# Autodesk Inventor assembly: CARRO
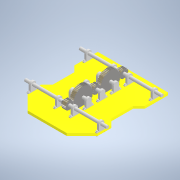
[picture p0: Inventor's stored thumbnail of the model, 180x180]
Saved by Autodesk Inventor 2021 (Build 250183000, 183)
## iProperties
Created: 2021-02-07
Part Number: CARRO
Document SubType Name: Assembly
Designer: rotje
Author: rotje
## Documents named in this file (5)
- C:\Users\rotje\Documents\Inventor\MSF\CARRO.iam
- C:\Users\rotje\Documents\Inventor\MSF\Base-soporte.iam
- C:\Users\rotje\Documents\Inventor\MSF\Eje-engrane.iam
- C:\Users\rotje\Documents\Inventor\MSF\Eje-engrane_chico.iam
- C:\Users\rotje\Documents\Inventor\MSF\Eje_Engrane-llanta.iam
## Components (6 placed, 4 different names)
1. Base-soporte:1 [sub-assembly] — Insertar:1, Insertar:2, Insertar:3, Coincidencia:1, Coincidencia:2, Coincidencia:3, Coincidencia:4
2. Eje-engrane:1 [sub-assembly] — Insertar:3, Nivelación:1, Tangente:3, Tangente:4, Rotación:3, Rotación:4
3. Eje-engrane:2 [sub-assembly] — Insertar:1, Nivelación:2, Tangente:1, Tangente:2, Rotación:1, Rotación:2
4. Eje-engrane_chico:1 [sub-assembly] — Insertar:2, Tangente:2, Tangente:3, Rotación:2, Rotación:3
5. Eje_Engrane-llanta:1 [sub-assembly] — Nivelación:1, Coincidencia:2, Tangente:4, Rotación:4
6. Eje_Engrane-llanta:2 [sub-assembly] — Nivelación:2, Coincidencia:3, Tangente:1, Rotación:1
## Relationships (17: Mate 4, Tangent 4, RelateRotation 4, Insert 3, Flush 2)
- Insertar:1: Base-soporte:1 ↔ Eje-engrane:2
- Insertar:2: Base-soporte:1 ↔ Eje-engrane_chico:1
- Insertar:3: Base-soporte:1 ↔ Eje-engrane:1
- Coincidencia:1 [Mate]: Base-soporte:1
- Nivelación:1 [Flush]: Eje-engrane:1 ↔ Eje_Engrane-llanta:1
- Nivelación:2 [Flush]: Eje-engrane:2 ↔ Eje_Engrane-llanta:2
- Coincidencia:2 [Mate]: Base-soporte:1 ↔ Eje_Engrane-llanta:1
- Coincidencia:3 [Mate]: Base-soporte:1 ↔ Eje_Engrane-llanta:2
- Tangente:1: Eje-engrane:2 ↔ Eje_Engrane-llanta:2
- Tangente:2: Eje-engrane:2 ↔ Eje-engrane_chico:1
- Tangente:3: Eje-engrane:1 ↔ Eje-engrane_chico:1
- Tangente:4: Eje-engrane:1 ↔ Eje_Engrane-llanta:1
- Rotación:1 [RelateRotation] (0.4 ul): Eje-engrane:2 ↔ Eje_Engrane-llanta:2
- Rotación:2 [RelateRotation] (2.5 ul): Eje-engrane:2 ↔ Eje-engrane_chico:1
- Rotación:3 [RelateRotation] (0.4 ul): Eje-engrane:1 ↔ Eje-engrane_chico:1
- Rotación:4 [RelateRotation] (2.5 ul): Eje-engrane:1 ↔ Eje_Engrane-llanta:1
- Coincidencia:4 [Mate]: Base-soporte:1
